# Autodesk Inventor assembly: DELL 1909Wf
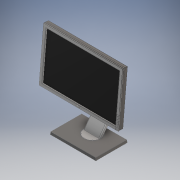
[picture p0: Inventor's stored thumbnail of the model, 180x180]
Saved by Autodesk Inventor 2017 SP1 (Build 210196100, 196)
## iProperties
Created: 2020-12-19
Part Number: DELL 1909Wf
Document SubType Name: Assembly
Designer: Napoleon
Author: Napoleon
## Documents named in this file (3)
- D:\PRYWATNE\PROJEKTY\POKÓJ\URZĄDZENIA PERYFERYJNE\DELL 1909Wf\DELL 1909Wf.iam
- D:\PRYWATNE\PROJEKTY\POKÓJ\URZĄDZENIA PERYFERYJNE\DELL 1909Wf\OBUDOWA TYLNA + PRZEDNIA + BLACHA ZE ZŁĄCZAMI.iam
- D:\PRYWATNE\PROJEKTY\POKÓJ\URZĄDZENIA PERYFERYJNE\DELL 1909Wf\PODSTAWA + STOJAK.iam
## Components (2 placed, 2 different names)
1. OBUDOWA TYLNA + PRZEDNIA + BLACHA ZE ZŁĄCZAMI:1 [sub-assembly] — Zestawiający:2, Równoległy:1, Zestawiający:3
2. PODSTAWA + STOJAK [sub-assembly] — Zestawiający:2, Równoległy:1, Zestawiający:3
## Relationships (3: Mate 2, Flush 1)
- Zestawiający:2 [Mate] (0.25 mm): OBUDOWA TYLNA + PRZEDNIA + BLACHA ZE ZŁĄCZAMI:1 ↔ PODSTAWA + STOJAK
- Równoległy:1 [Flush]: OBUDOWA TYLNA + PRZEDNIA + BLACHA ZE ZŁĄCZAMI:1 ↔ PODSTAWA + STOJAK
- Zestawiający:3 [Mate] (0.01 mm): OBUDOWA TYLNA + PRZEDNIA + BLACHA ZE ZŁĄCZAMI:1 ↔ PODSTAWA + STOJAK
